# Autodesk Inventor assembly: Assembly4
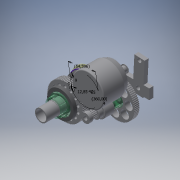
[picture p0: Inventor's stored thumbnail of the model, 180x180]
Saved by Autodesk Inventor 2018.1 (Build 221171000, 171)
## iProperties
Created: 2022-06-29
Part Number: Assembly4
Document SubType Name: Assembly
Designer: Bureau
Author: Bureau
## Documents named in this file (6)
- C:\Users\mouta\GoogleDrive\Manu\USINAGE\MoteurVelo\Assembly4.iam
- C:\Users\mouta\GoogleDrive\Manu\USINAGE\MoteurVelo\Arbre secondaire\Assembly3.iam
- C:\Users\mouta\GoogleDrive\Manu\USINAGE\MoteurVelo\Arbre primaire\Assembly1.iam
- C:\Users\mouta\GoogleDrive\Manu\USINAGE\MoteurVelo\Corps\plaque 1.ipt
- C:\Users\mouta\GoogleDrive\Manu\USINAGE\MoteurVelo\Moteur\moteur.iam
- C:\Users\mouta\GoogleDrive\Manu\USINAGE\MoteurVelo\Corps\plaque 2.ipt
## Components (5 placed, 5 different names)
1. Assembly1:1 [sub-assembly] — Mate:1, Mate:3
2. plaque 1:1 — Mate:1, Mate:3, Mate:4, Mate:5, Flush:1, Angle:1, Mate:9
3. Assembly3:1 [sub-assembly] — Mate:4, Mate:5
4. moteur:1 [sub-assembly] — Mate:7, Mate:8
5. plaque 2:1 — Flush:1, Mate:7, Mate:8, Angle:1, Mate:9
## Relationships (9: Mate 7, Flush 1, Angle 1)
- Mate:1: Assembly1:1 ↔ plaque 1:1
- Mate:3: Assembly1:1 ↔ plaque 1:1
- Mate:4 (33 mm): plaque 1:1 ↔ Assembly3:1
- Mate:5: plaque 1:1 ↔ Assembly3:1
- Flush:1: plaque 1:1 ↔ plaque 2:1
- Mate:7: moteur:1 ↔ plaque 2:1
- Mate:8 (28 mm): moteur:1 ↔ plaque 2:1
- Angle:1 (3 deg): plaque 1:1 ↔ plaque 2:1
- Mate:9: plaque 1:1 ↔ plaque 2:1
